# Autodesk Inventor assembly: Clamp with Piston Assembly
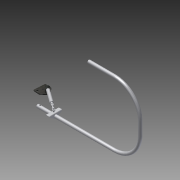
[picture p0: Inventor's stored thumbnail of the model, 180x180]
Saved by Autodesk Inventor 2014 (Build 180170000, 170)
## iProperties
Created: 2014-01-12
Part Number: Clamp with Piston Assembly
Document SubType Name: Assembly
Designer: Michael
Author: Michael
## Documents named in this file (5)
- C:\Users\Michael\Documents\Robotics\2014 Season\Collector\Clamp with Piston Assembly.iam
- C:\Users\Michael\Documents\Robotics\2014 Season\Collector\Metal Pipe Clamp.ipt
- C:\Users\Michael\Documents\Robotics\2014 Season\Collector\Pipe to Gas Spring Connector (9417K91).ipt
- C:\Users\Michael\Documents\Robotics\2014 Season\Collector\Gas Spring Support (9417K910).ipt
- C:\Users\Michael\Documents\Robotics\2014 Season\Collector\Gas Spring (9417K161).ipt
## Components (4 placed, 4 different names)
1. Metal Pipe Clamp:1 — Mate:1, Mate:2
2. Pipe to Gas Spring Connector (9417K91):1 — Mate:1, Mate:2, Insert:4
3. Gas Spring Support (9417K910):1 — Insert:3
4. Gas Spring (9417K161):1 — Insert:3, Insert:4
## Relationships (4: Mate 2, Insert 2)
- Mate:1: Metal Pipe Clamp:1 ↔ Pipe to Gas Spring Connector (9417K91):1
- Mate:2: Metal Pipe Clamp:1 ↔ Pipe to Gas Spring Connector (9417K91):1
- Insert:3: Gas Spring Support (9417K910):1 ↔ Gas Spring (9417K161):1
- Insert:4 (3.175 mm): Pipe to Gas Spring Connector (9417K91):1 ↔ Gas Spring (9417K161):1
